# Autodesk Inventor assembly: Con_Vibraciones
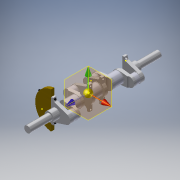
[picture p0: Inventor's stored thumbnail of the model, 180x180]
Saved by Autodesk Inventor 2019 (Build 230136000, 136)
## iProperties
Created: 2019-07-01
Part Number: Con_Vibraciones
Document SubType Name: Assembly
Designer: Oscar Rojas
Author: Oscar Rojas
## Documents named in this file (4)
- E:\OSCAR\UNAL\6to SEMESTRE\Principios de dinámica\Proyectos\Proyecto 2\Mio\Con_Vibraciones.iam
- E:\OSCAR\UNAL\6to SEMESTRE\Principios de dinámica\Proyectos\Proyecto 2\Mio\cigueñal.ipt
- E:\OSCAR\UNAL\6to SEMESTRE\Principios de dinámica\Proyectos\Proyecto 2\Mio\ContrapesoGrande1.ipt
- E:\OSCAR\UNAL\6to SEMESTRE\Principios de dinámica\Proyectos\Proyecto 2\Mio\Pasador.ipt
## Components (4 placed, 3 different names)
1. cigueñal:1 — Rotational:1
2. ContrapesoGrande1:1 — Rotational:1, Insert:1, Insert:2
3. Pasador:1 — Insert:2
4. Pasador:2 — Insert:1
## Relationships (3: Insert 2, RevoluteJoint 1)
- Rotational:1 [RevoluteJoint]: cigueñal:1 ↔ ContrapesoGrande1:1
- Insert:1 (-30 mm): ContrapesoGrande1:1 ↔ Pasador:2
- Insert:2 (-30 mm): ContrapesoGrande1:1 ↔ Pasador:1
